# Autodesk Inventor assembly: A1-19027-100-00 Spool RD-51-L-585-1
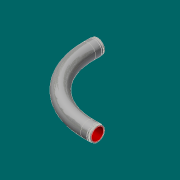
[picture p0: Inventor's stored thumbnail of the model, 180x180]
Saved by Autodesk Inventor 2017.3 (Build 213256000, 256)
## iProperties
Created: 2019-06-26
Part Number: A1-19027-100-00 Spool RD-51-L-585-1
Document SubType Name: Weldment
Designer: Graeme_Van_Dongen
Weld Material: Steel, Mild, Welded
Mass: 9.09415e+06 g
Surface Area: 805156 cm^2
Volume: 1.21858e+06 cm^3
Density: 7.46291 g/cm^3
Author: Graeme_Van_Dongen
## Documents named in this file (4)
- N:\A1 - Projects\A1-19\A1-19027--Syncrude Aurora Train 2 reducer and elbow\A1-19027-100-00 Spool RD-51-L-585-1.iam
- N:\A1 - Projects\A1-19\A1-19027--Syncrude Aurora Train 2 reducer and elbow\A1-19027-100-01 36in elbow.ipt
- N:\A1 - Projects\A1-19\A1-19027--Syncrude Aurora Train 2 reducer and elbow\A1-19027-100-xx 32in Type B victaulic ring.ipt
- N:\A1 - Projects\A1-19\A1-19027--Syncrude Aurora Train 2 reducer and elbow\A1-19027-100-xx HCWI elbow.ipt
## Components (4 placed, 3 different names)
1. A1-19027-100-01 36in elbow:1 — Insert:1, Angle:1, Insert:2, Angle:2, Flush:1, Mate:1, Angle:3
2. A1-19027-100-xx 32in Type B victaulic ring:1 — Insert:1, Angle:1
3. A1-19027-100-xx 32in Type B victaulic ring:2 — Insert:2, Angle:2
4. A1-19027-100-xx HCWI elbow:1 — Flush:1, Mate:1, Angle:3
## Relationships (7: Angle 3, Insert 2, Flush 1, Mate 1)
- Insert:1 (2.3813 mm): A1-19027-100-01 36in elbow:1 ↔ A1-19027-100-xx 32in Type B victaulic ring:1
- Angle:1 (0 deg): A1-19027-100-01 36in elbow:1 ↔ A1-19027-100-xx 32in Type B victaulic ring:1
- Insert:2 (2.3813 mm): A1-19027-100-01 36in elbow:1 ↔ A1-19027-100-xx 32in Type B victaulic ring:2
- Angle:2 (0 deg): A1-19027-100-01 36in elbow:1 ↔ A1-19027-100-xx 32in Type B victaulic ring:2
- Flush:1: A1-19027-100-01 36in elbow:1 ↔ A1-19027-100-xx HCWI elbow:1
- Mate:1: A1-19027-100-01 36in elbow:1 ↔ A1-19027-100-xx HCWI elbow:1
- Angle:3 (0 deg): A1-19027-100-01 36in elbow:1 ↔ A1-19027-100-xx HCWI elbow:1
